# Autodesk Inventor assembly: Máquina boca de pescado automatizada
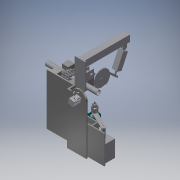
[picture p0: Inventor's stored thumbnail of the model, 180x180]
Saved by Autodesk Inventor 2018 (Build 220112000, 112)
## iProperties
Created: 2021-07-05
Part Number: Máquina boca de pescado automatizada
Material: Genérico
Document SubType Name: Assembly
Designer: GABRIEL
Author: GABRIEL
## Documents named in this file (28)
- C:\Users\GABRIEL\Documents\Gabriel\UNAL\SEMESTRE XI\Automatización de PM\Proyecto\Maquina de boca de pescado\Máquina boca de pescado automatizada.iam
- C:\Users\GABRIEL\Documents\Gabriel\Modelados\Placa1.ipt
- C:\Users\GABRIEL\Documents\Gabriel\UNAL\SEMESTRE XI\Automatización de PM\Proyecto\Maquina de boca de pescado\Base.ipt
- C:\Users\GABRIEL\Documents\Gabriel\UNAL\SEMESTRE XI\Automatización de PM\Proyecto\Maquina de boca de pescado\Posicionador.ipt
- C:\Users\GABRIEL\Documents\Gabriel\UNAL\SEMESTRE XI\Automatización de PM\Proyecto\Maquina de boca de pescado\Rodamiento.iam
- C:\Users\GABRIEL\Documents\Gabriel\UNAL\SEMESTRE XI\Automatización de PM\Proyecto\Maquina de boca de pescado\Soporte_rods.ipt
- C:\Users\GABRIEL\Documents\Gabriel\UNAL\SEMESTRE XI\Automatización de PM\Proyecto\Maquina de boca de pescado\eje.ipt
- C:\Users\GABRIEL\Documents\Gabriel\UNAL\SEMESTRE XI\Automatización de PM\Proyecto\Maquina de boca de pescado\spindle.ipt
- C:\Users\GABRIEL\Documents\Gabriel\UNAL\SEMESTRE XI\Automatización de PM\Proyecto\Maquina de boca de pescado\anclaje.ipt
- C:\Users\GABRIEL\Documents\Gabriel\UNAL\SEMESTRE XI\Automatización de PM\Proyecto\Maquina de boca de pescado\ancla.ipt
- C:\Users\GABRIEL\Documents\Gabriel\UNAL\SEMESTRE XI\Automatización de PM\Proyecto\Maquina de boca de pescado\ancla_tornillo.ipt
- C:\Users\GABRIEL\Documents\Gabriel\UNAL\SEMESTRE XI\Automatización de PM\Proyecto\Maquina de boca de pescado\sujetador.ipt
- C:\Users\GABRIEL\Documents\Gabriel\UNAL\SEMESTRE XI\Automatización de PM\Proyecto\Maquina de boca de pescado\din_912-m20x1_5-200-10_9.ipt
- C:\Users\GABRIEL\Documents\Gabriel\UNAL\SEMESTRE XI\Automatización de PM\Proyecto\Maquina de boca de pescado\encaje.ipt
- C:\Users\GABRIEL\Documents\Gabriel\UNAL\SEMESTRE XI\Automatización de PM\Proyecto\Maquina de boca de pescado\22200-0580308315.ipt
- C:\Users\GABRIEL\Documents\Gabriel\UNAL\SEMESTRE XI\Automatización de PM\Proyecto\Maquina de boca de pescado\motor_cml-30.ipt
- C:\Users\GABRIEL\Documents\Gabriel\UNAL\SEMESTRE XI\Automatización de PM\Proyecto\Maquina de boca de pescado\Tubo_ensayo.ipt
- C:\Users\GABRIEL\Documents\Gabriel\UNAL\SEMESTRE XI\Automatización de PM\Proyecto\Maquina de boca de pescado\Varilla_suj.ipt
- C:\Users\GABRIEL\Documents\Gabriel\UNAL\SEMESTRE XI\Automatización de PM\Proyecto\Maquina de boca de pescado\base_motor.ipt
- C:\Users\GABRIEL\Documents\Gabriel\UNAL\SEMESTRE XI\Automatización de PM\Proyecto\Maquina de boca de pescado\Riel.ipt
- C:\Users\GABRIEL\Documents\Gabriel\UNAL\SEMESTRE XI\Automatización de PM\Proyecto\Maquina de boca de pescado\Carro_riel.ipt
- C:\Users\GABRIEL\Documents\Gabriel\UNAL\SEMESTRE XI\Automatización de PM\Proyecto\Maquina de boca de pescado\base_motor_taladro.ipt
- C:\Users\GABRIEL\Documents\Gabriel\UNAL\SEMESTRE XI\Automatización de PM\Proyecto\Maquina de boca de pescado\Motor_suj.iam
- C:\Users\GABRIEL\Documents\Gabriel\UNAL\SEMESTRE XI\Automatización de PM\Proyecto\Maquina de boca de pescado\M_taladro.ipt
- C:\Users\GABRIEL\Documents\Gabriel\UNAL\SEMESTRE XI\Automatización de PM\Proyecto\Maquina de boca de pescado\union_cil_tal.ipt
- C:\Users\GABRIEL\Documents\Gabriel\UNAL\SEMESTRE XI\Automatización de PM\Proyecto\Maquina de boca de pescado\Cilindro.ipt
- C:\Users\GABRIEL\Documents\Gabriel\UNAL\SEMESTRE XI\Automatización de PM\Proyecto\Maquina de boca de pescado\cilindro_tal.ipt
- C:\Users\GABRIEL\Documents\Gabriel\UNAL\SEMESTRE XI\Automatización de PM\Proyecto\Maquina de boca de pescado\Sierra.iam
## Components (48 placed, 27 different names)
1. Base:1 — Nivelación:1, Nivelación:2, Nivelación:3, Coincidencia:75, Ángulo:4, Coincidencia:84, Coincidencia:85, Coincidencia:86, Coincidencia:87, Coincidencia:88, Coincidencia:89, Coincidencia:90, Coincidencia:91, Nivelación:38, Coincidencia:100, Coincidencia:101
2. Soporte:1 — Nivelación:1, Nivelación:2, Coincidencia:3, Coincidencia:16, Coincidencia:62, Coincidencia:65, Coincidencia:84
3. Soporte:2 — Nivelación:3, Coincidencia:3, Tangente:1, Tangente:2, Coincidencia:68, Coincidencia:85
4. Posicionador:1 — Coincidencia:8, Nivelación:6, Nivelación:7, Coincidencia:75, Ángulo:4, Coincidencia:76, Coincidencia:90, Coincidencia:92, Coincidencia:98, Nivelación:37
5. Rodamiento:1 [sub-assembly] — Coincidencia:9, Nivelación:8, Nivelación:21, Insertar:6
6. Soporte_rods:1 — Coincidencia:8, Nivelación:6, Nivelación:7, Coincidencia:9, Nivelación:8, Nivelación:21, Coincidencia:77, Nivelación:22, Nivelación:23, Coincidencia:78, Nivelación:24, Nivelación:25
7. eje:1 — Coincidencia:13, Coincidencia:14, Rotación:1, Insertar:6, Insertar:7, Coincidencia:96
8. spindle:1 — Coincidencia:13, Coincidencia:14, Rotación:1, Coincidencia:97
9. anclaje:1 — Coincidencia:16, Coincidencia:17, Coincidencia:18, Coincidencia:19, Coincidencia:20, Coincidencia:21, Coincidencia:22, Ángulo:2, Coincidencia:26, Ángulo:3, Coincidencia:61, Coincidencia:62, Coincidencia:63, Coincidencia:67, Coincidencia:86
10. ancla:1 — Coincidencia:17, Coincidencia:18, Coincidencia:23, Coincidencia:25
11. ancla:2 — Coincidencia:19, Coincidencia:20, Coincidencia:24
12. ancla_tornillo:1 — Coincidencia:21, Coincidencia:22, Coincidencia:60
13. sujetador:1 — Insertar:2, Insertar:3, Coincidencia:25, Nivelación:13, Coincidencia:87
14. din_912-m20x1_5-200-10_9:1 — Insertar:3, Coincidencia:24, Insertar:5
15. din_912-m20x1_5-200-10_9:2 — Insertar:2, Coincidencia:23, Insertar:4
16. encaje:1 — Insertar:4, Ángulo:2, Coincidencia:26, Coincidencia:27, Coincidencia:30, Coincidencia:31, Coincidencia:49, Coincidencia:52, Coincidencia:54
17. encaje:2 — Insertar:5, Ángulo:3, Coincidencia:36, Coincidencia:50, Coincidencia:53
18. 22200-0580308315:1 — Coincidencia:27, Coincidencia:28, Coincidencia:29, Coincidencia:30, Coincidencia:31, Coincidencia:51
19. 22200-0580308315:2 — Coincidencia:28, Coincidencia:29, Coincidencia:32, Coincidencia:33, Tangente:8, Tangente:9
20. 22200-0580308315:3 — Coincidencia:32, Coincidencia:33, Coincidencia:34, Coincidencia:35, Tangente:10
21. 22200-0580308315:5 — Coincidencia:34, Coincidencia:35, Coincidencia:36
22. 22200-0580308315:6 — Coincidencia:52, Coincidencia:54, Coincidencia:55
23. 22200-0580308315:7 — Tangente:4, Tangente:5
24. 22200-0580308315:8 — Tangente:3
25. 22200-0580308315:9 — Coincidencia:53
26. 22200-0580308315:10 — Coincidencia:49, Coincidencia:51, Coincidencia:55
27. 22200-0580308315:11 — Tangente:6
28. 22200-0580308315:12 — Tangente:7, Tangente:11
29. 22200-0580308315:13 — Coincidencia:50
30. motor_cml-30:1 — Coincidencia:76, Coincidencia:91, Coincidencia:92
31. Tubo_ensayo:1 — Tangente:1, Tangente:2, Tangente:3, Tangente:4, Tangente:5, Tangente:6, Tangente:7, Tangente:8, Tangente:9, Tangente:10, Tangente:11
32. Varilla_suj:1 — Coincidencia:60, Coincidencia:61, Nivelación:13, Coincidencia:94
33. base_motor:1 — Coincidencia:73, Nivelación:18, Nivelación:19, Nivelación:20, Coincidencia:93, Nivelación:33, Nivelación:34
34. Riel:1 — Coincidencia:63, Coincidencia:65, Coincidencia:69, Coincidencia:70, Nivelación:14, Nivelación:15, Coincidencia:88
35. Riel:2 — Coincidencia:67, Coincidencia:68, Coincidencia:71, Coincidencia:72, Nivelación:16, Nivelación:17, Coincidencia:89
36. Carro_riel:1 — Coincidencia:71, Coincidencia:72, Nivelación:16, Nivelación:17, Nivelación:20
37. Carro_riel:2 — Coincidencia:69, Coincidencia:70, Nivelación:14, Nivelación:15, Coincidencia:73, Nivelación:18, Nivelación:19
38. Riel:3 — Coincidencia:78, Nivelación:24, Nivelación:25, Coincidencia:81, Coincidencia:82, Nivelación:28, Nivelación:29
39. Riel:4 — Coincidencia:77, Nivelación:22, Nivelación:23, Coincidencia:79, Coincidencia:80, Nivelación:26, Nivelación:27
40. Carro_riel:3 — Coincidencia:81, Coincidencia:82, Nivelación:28, Nivelación:29, Nivelación:30, Nivelación:31
41. Carro_riel:4 — Coincidencia:79, Coincidencia:80, Nivelación:26, Nivelación:27, Coincidencia:83, Nivelación:32
42. base_motor_taladro:1 — Coincidencia:83, Nivelación:30, Nivelación:31, Nivelación:32, Coincidencia:95, Nivelación:35, Nivelación:36
43. Motor_suj:1 [sub-assembly] — Coincidencia:93, Nivelación:33, Nivelación:34, Coincidencia:94
44. M_taladro:1 — Coincidencia:95, Nivelación:35, Insertar:7, Nivelación:36, Ángulo:6
45. union_cil_tal:1 — Coincidencia:96, Ángulo:6, Coincidencia:97, Insertar:8
46. Cilindro:1 — Coincidencia:98, Coincidencia:99, Nivelación:37
47. cilindro_tal:1 — Insertar:8, Coincidencia:99
48. Sierra:1 [sub-assembly] — Nivelación:38, Coincidencia:100, Coincidencia:101
## Relationships (139: Mate 84, Flush 32, Tangent 11, Insert 7, Angle 4, RelateRotation 1)
- Nivelación:1 [Flush] (10 mm): Base:1 ↔ Soporte:1
- Nivelación:2 [Flush] (-10 mm): Base:1 ↔ Soporte:1
- Nivelación:3 [Flush] (10 mm): Base:1 ↔ Soporte:2
- Coincidencia:3 [Mate] (100 mm): Soporte:1 ↔ Soporte:2
- Coincidencia:8 [Mate]: Posicionador:1 ↔ Soporte_rods:1
- Nivelación:6 [Flush]: Posicionador:1 ↔ Soporte_rods:1
- Nivelación:7 [Flush]: Posicionador:1 ↔ Soporte_rods:1
- Coincidencia:9 [Mate]: Rodamiento:1 ↔ Soporte_rods:1
- Nivelación:8 [Flush]: Rodamiento:1 ↔ Soporte_rods:1
- Coincidencia:13 [Mate]: eje:1 ↔ spindle:1
- Coincidencia:14 [Mate]: eje:1 ↔ spindle:1
- Rotación:1 [RelateRotation] (1 ul): eje:1 ↔ spindle:1
- Coincidencia:16 [Mate] (10 mm): Soporte:1 ↔ anclaje:1
- Coincidencia:17 [Mate]: anclaje:1 ↔ ancla:1
- Coincidencia:18 [Mate]: anclaje:1 ↔ ancla:1
- Coincidencia:19 [Mate]: anclaje:1 ↔ ancla:2
- Coincidencia:20 [Mate]: anclaje:1 ↔ ancla:2
- Coincidencia:21 [Mate]: anclaje:1 ↔ ancla_tornillo:1
- Coincidencia:22 [Mate]: anclaje:1 ↔ ancla_tornillo:1
- Insertar:2: sujetador:1 ↔ din_912-m20x1_5-200-10_9:2
- Insertar:3: sujetador:1 ↔ din_912-m20x1_5-200-10_9:1
- Coincidencia:23 [Mate]: ancla:1 ↔ din_912-m20x1_5-200-10_9:2
- Coincidencia:24 [Mate]: ancla:2 ↔ din_912-m20x1_5-200-10_9:1
- Coincidencia:25 [Mate]: ancla:1 ↔ sujetador:1
- Insertar:4 (-10 mm): din_912-m20x1_5-200-10_9:2 ↔ encaje:1
- Ángulo:2 [Angle] (0 deg): anclaje:1 ↔ encaje:1
- Coincidencia:26 [Mate]: anclaje:1 ↔ encaje:1
- Insertar:5 (-15 mm): din_912-m20x1_5-200-10_9:1 ↔ encaje:2
- Ángulo:3 [Angle] (0 deg): anclaje:1 ↔ encaje:2
- Coincidencia:27 [Mate]: encaje:1 ↔ 22200-0580308315:1
- Coincidencia:28 [Mate]: 22200-0580308315:1 ↔ 22200-0580308315:2
- Coincidencia:29 [Mate]: 22200-0580308315:1 ↔ 22200-0580308315:2
- Coincidencia:30 [Mate]: encaje:1 ↔ 22200-0580308315:1
- Coincidencia:31 [Mate]: encaje:1 ↔ 22200-0580308315:1
- Coincidencia:32 [Mate]: 22200-0580308315:2 ↔ 22200-0580308315:3
- Coincidencia:33 [Mate]: 22200-0580308315:2 ↔ 22200-0580308315:3
- Coincidencia:34 [Mate]: 22200-0580308315:3 ↔ 22200-0580308315:5
- Coincidencia:35 [Mate]: 22200-0580308315:3 ↔ 22200-0580308315:5
- Coincidencia:36 [Mate]: encaje:2 ↔ 22200-0580308315:5
- [Mate]: 22200-0580308315:6 ↔ 22200-0580308315:7
- [Mate]: 22200-0580308315:6 ↔ 22200-0580308315:7
- [Mate]: 22200-0580308315:7 ↔ 22200-0580308315:8
- [Mate]: 22200-0580308315:7 ↔ 22200-0580308315:8
- [Mate]: 22200-0580308315:8 ↔ 22200-0580308315:9
- [Mate]: 22200-0580308315:8 ↔ 22200-0580308315:9
- [Mate]: 22200-0580308315:10 ↔ 22200-0580308315:11
- [Mate]: 22200-0580308315:10 ↔ 22200-0580308315:11
- [Mate]: 22200-0580308315:11 ↔ 22200-0580308315:12
- [Mate]: 22200-0580308315:11 ↔ 22200-0580308315:12
- [Mate]: 22200-0580308315:12 ↔ 22200-0580308315:13
- [Mate]: 22200-0580308315:12 ↔ 22200-0580308315:13
- Coincidencia:49 [Mate]: encaje:1 ↔ 22200-0580308315:10
- Coincidencia:50 [Mate]: encaje:2 ↔ 22200-0580308315:13
- Coincidencia:51 [Mate]: 22200-0580308315:1 ↔ 22200-0580308315:10
- Coincidencia:52 [Mate]: encaje:1 ↔ 22200-0580308315:6
- Coincidencia:53 [Mate]: encaje:2 ↔ 22200-0580308315:9
- Coincidencia:54 [Mate]: encaje:1 ↔ 22200-0580308315:6
- Coincidencia:55 [Mate]: 22200-0580308315:6 ↔ 22200-0580308315:10
- Tangente:1: Soporte:2 ↔ Tubo_ensayo:1
- Tangente:2: Soporte:2 ↔ Tubo_ensayo:1
- Tangente:3: 22200-0580308315:8 ↔ Tubo_ensayo:1
- Tangente:4: 22200-0580308315:7 ↔ Tubo_ensayo:1
- Tangente:5: 22200-0580308315:7 ↔ Tubo_ensayo:1
- Tangente:6: 22200-0580308315:11 ↔ Tubo_ensayo:1
- Tangente:7: 22200-0580308315:12 ↔ Tubo_ensayo:1
- Tangente:8: 22200-0580308315:2 ↔ Tubo_ensayo:1
- Tangente:9: 22200-0580308315:2 ↔ Tubo_ensayo:1
- Tangente:10: 22200-0580308315:3 ↔ Tubo_ensayo:1
- Tangente:11: 22200-0580308315:12 ↔ Tubo_ensayo:1
- Coincidencia:60 [Mate]: ancla_tornillo:1 ↔ Varilla_suj:1
- Coincidencia:61 [Mate]: anclaje:1 ↔ Varilla_suj:1
- Nivelación:13 [Flush] (-50 mm): sujetador:1 ↔ Varilla_suj:1
- Coincidencia:62 [Mate] (10 mm): Soporte:1 ↔ anclaje:1
- Coincidencia:63 [Mate] (9 mm): anclaje:1 ↔ Riel:1
- Coincidencia:65 [Mate] (180 mm): Soporte:1 ↔ Riel:1
- Coincidencia:67 [Mate] (9 mm): anclaje:1 ↔ Riel:2
- Coincidencia:68 [Mate] (180 mm): Soporte:2 ↔ Riel:2
- Coincidencia:69 [Mate]: Riel:1 ↔ Carro_riel:2
- Coincidencia:70 [Mate]: Riel:1 ↔ Carro_riel:2
- Coincidencia:71 [Mate]: Riel:2 ↔ Carro_riel:1
- Coincidencia:72 [Mate]: Riel:2 ↔ Carro_riel:1
- Nivelación:14 [Flush]: Riel:1 ↔ Carro_riel:2
- Nivelación:15 [Flush]: Riel:1 ↔ Carro_riel:2
- Nivelación:16 [Flush]: Riel:2 ↔ Carro_riel:1
- Nivelación:17 [Flush]: Riel:2 ↔ Carro_riel:1
- Coincidencia:73 [Mate]: base_motor:1 ↔ Carro_riel:2
- Nivelación:18 [Flush]: base_motor:1 ↔ Carro_riel:2
- Nivelación:19 [Flush] (15 mm): base_motor:1 ↔ Carro_riel:2
- Nivelación:20 [Flush] (15 mm): base_motor:1 ↔ Carro_riel:1
- Coincidencia:75 [Mate]: Base:1 ↔ Posicionador:1
- Ángulo:4 [Angle] (0 deg): Base:1 ↔ Posicionador:1
- Coincidencia:76 [Mate]: Posicionador:1 ↔ motor_cml-30:1
- Nivelación:21 [Flush]: Rodamiento:1 ↔ Soporte_rods:1
- Insertar:6: Rodamiento:1 ↔ eje:1
- Coincidencia:77 [Mate]: Soporte_rods:1 ↔ Riel:4
- Nivelación:22 [Flush]: Soporte_rods:1 ↔ Riel:4
- Nivelación:23 [Flush] (10 mm): Soporte_rods:1 ↔ Riel:4
- Coincidencia:78 [Mate]: Soporte_rods:1 ↔ Riel:3
- Nivelación:24 [Flush] (-10 mm): Soporte_rods:1 ↔ Riel:3
- Nivelación:25 [Flush]: Soporte_rods:1 ↔ Riel:3
- Coincidencia:79 [Mate]: Riel:4 ↔ Carro_riel:4
- Coincidencia:80 [Mate]: Riel:4 ↔ Carro_riel:4
- Nivelación:26 [Flush]: Riel:4 ↔ Carro_riel:4
- Nivelación:27 [Flush]: Riel:4 ↔ Carro_riel:4
- Coincidencia:81 [Mate]: Riel:3 ↔ Carro_riel:3
- Coincidencia:82 [Mate]: Riel:3 ↔ Carro_riel:3
- Nivelación:28 [Flush]: Riel:3 ↔ Carro_riel:3
- Nivelación:29 [Flush]: Riel:3 ↔ Carro_riel:3
- Coincidencia:83 [Mate]: Carro_riel:4 ↔ base_motor_taladro:1
- Nivelación:30 [Flush]: Carro_riel:3 ↔ base_motor_taladro:1
- Nivelación:31 [Flush] (-15 mm): Carro_riel:3 ↔ base_motor_taladro:1
- Nivelación:32 [Flush] (-15 mm): Carro_riel:4 ↔ base_motor_taladro:1
- Coincidencia:84 [Mate]: Base:1 ↔ Soporte:1
- Coincidencia:85 [Mate]: Base:1 ↔ Soporte:2
- Coincidencia:86 [Mate]: Base:1 ↔ anclaje:1
- Coincidencia:87 [Mate]: Base:1 ↔ sujetador:1
- Coincidencia:88 [Mate]: Base:1 ↔ Riel:1
- Coincidencia:89 [Mate]: Base:1 ↔ Riel:2
- Coincidencia:90 [Mate]: Base:1 ↔ Posicionador:1
- Coincidencia:91 [Mate]: Base:1 ↔ motor_cml-30:1
- Coincidencia:92 [Mate]: Posicionador:1 ↔ motor_cml-30:1
- Coincidencia:93 [Mate]: base_motor:1 ↔ Motor_suj:1
- Nivelación:33 [Flush] (35 mm): base_motor:1 ↔ Motor_suj:1
- Nivelación:34 [Flush] (30 mm): base_motor:1 ↔ Motor_suj:1
- Coincidencia:94 [Mate]: Varilla_suj:1 ↔ Motor_suj:1
- Coincidencia:95 [Mate]: base_motor_taladro:1 ↔ M_taladro:1
- Nivelación:35 [Flush] (31 mm): base_motor_taladro:1 ↔ M_taladro:1
- Insertar:7 (-20 mm): eje:1 ↔ M_taladro:1
- Nivelación:36 [Flush] (5 mm): base_motor_taladro:1 ↔ M_taladro:1
- Coincidencia:96 [Mate]: eje:1 ↔ union_cil_tal:1
- Ángulo:6 [Angle] (0 deg): M_taladro:1 ↔ union_cil_tal:1
- Coincidencia:97 [Mate]: spindle:1 ↔ union_cil_tal:1
- Insertar:8: union_cil_tal:1 ↔ cilindro_tal:1
- Coincidencia:98 [Mate]: Posicionador:1 ↔ Cilindro:1
- Coincidencia:99 [Mate]: Cilindro:1 ↔ cilindro_tal:1
- Nivelación:37 [Flush] (10 mm): Posicionador:1 ↔ Cilindro:1
- Nivelación:38 [Flush]: Base:1 ↔ Sierra:1
- Coincidencia:100 [Mate]: Base:1 ↔ Sierra:1
- Coincidencia:101 [Mate]: Base:1 ↔ Sierra:1
## Named parameters: d77_d73 = 0 mm, d78_d74 = 0 mm, d79_d75 = 0 mm, d80_d64 = 0 mm, d81_d65 = 0 mm, d82_d72 = 0 mm, d83_d73 = 0 mm, d84_d74 = 0 mm, d85_d75 = 0 mm, d86_d64 = 0 mm, d87_d65 = 0 mm, d88_d72 = 0 mm
